# Autodesk Inventor assembly: Main assembly
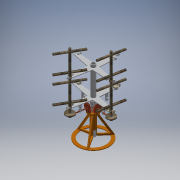
[picture p0: Inventor's stored thumbnail of the model, 180x180]
Saved by Autodesk Inventor 2018.1 (Build 221171000, 171)
## iProperties
Created: 2017-09-02
Part Number: Main assembly
Document SubType Name: Assembly
Designer: ToreDenStore
Author: ToreDenStore
## Documents named in this file (5)
- C:\Users\ToreDenStore\Documents\Inventor\VAWT3DPrint\Main assembly.iam
- C:\Users\ToreDenStore\Documents\Inventor\VAWT3DPrint\Base.ipt
- C:\Users\ToreDenStore\Documents\Inventor\VAWT3DPrint\Center beam.ipt
- C:\Users\ToreDenStore\Documents\Inventor\VAWT3DPrint\GearConnector.ipt
- C:\Users\ToreDenStore\Documents\Inventor\VAWT3DPrint\Sailbeam.ipt
## Components (6 placed, 4 different names)
1. Base:1 — Rotation:1, Rotational:1
2. Center beam:1 — Rotational:1, Rotational:2, Rotational:3, Rotational:4, Rotational:5
3. GearConnector:1 — Rotation:1, Rotation:2, Rotational:2
4. Sailbeam:1 — Rotation:2, Rotational:3
5. GearConnector:2 — Rotational:4
6. Sailbeam:2 — Rotational:5
## Relationships (7: RevoluteJoint 5, RelateRotation 2)
- Rotation:1 [RelateRotation] (0.8 ul): Base:1 ↔ GearConnector:1
- Rotation:2 [RelateRotation] (4.5 ul): GearConnector:1 ↔ Sailbeam:1
- Rotational:1 [RevoluteJoint]: Base:1 ↔ Center beam:1
- Rotational:2 [RevoluteJoint]: Center beam:1 ↔ GearConnector:1
- Rotational:3 [RevoluteJoint]: Center beam:1 ↔ Sailbeam:1
- Rotational:4 [RevoluteJoint]: Center beam:1 ↔ GearConnector:2
- Rotational:5 [RevoluteJoint]: Center beam:1 ↔ Sailbeam:2
